# Autodesk Inventor assembly: LIA0004 XILINX SHELF ASSY
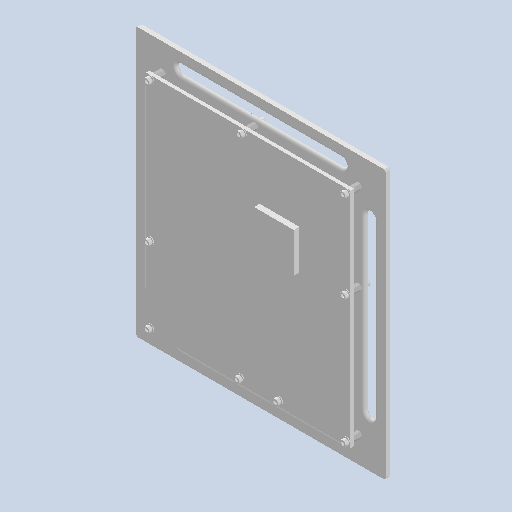
[picture p0: Inventor's stored thumbnail of the model, 512x512]
Saved by Autodesk Inventor 2023 (Build 270158000, 158)
## iProperties
Created: 2023-04-03
Part Number: LIA0004 XILINX SHELF ASSY
Document SubType Name: Assembly
Designer: Louis
Author: Louis
## Documents named in this file (7)
- D:\Louis\Documents\Inventor\Interferometry\LIA0004-XILINX SHELF ASSY.iam
- D:\Louis\Documents\Inventor\Interferometry\LI0009-XILINX SHELF.ipt
- D:\Louis\Documents\Inventor\Interferometry\XILINX BOARD FOOTPRINT.ipt
- D:\Louis\Documents\Inventor\Interferometry\ACCU HHTPS-M3-5-8-S-Z.ipt
- D:\Louis\Documents\Inventor\Interferometry\M3 WASHER.ipt
- D:\Louis\Documents\Inventor\Interferometry\M3 X 6.ipt
- D:\Louis\Documents\Inventor\Interferometry\XCZU48DR-FFVE1156 DIE.ipt
## Components (48 placed, 6 different names)
1. LI0009-XILINX SHELF:1 — Mate:1, Mate:2, Mate:3, Mate:4, Insert:1, Insert:2, Insert:3, Insert:4, Insert:5, Insert:6, Insert:7, Insert:8, Angle:1, Angle:2, Angle:3, Angle:4, Angle:5, Angle:6, Angle:7, Angle:8, Angle:9, Insert:27, Insert:28, Insert:29, Insert:30, Insert:31, Insert:32, Insert:33, Insert:34, Insert:35
2. XILINX BOARD FOOTPRINT:1 — Insert:9, Insert:10, Insert:11, Insert:12, Insert:13, Insert:14, Insert:15, Insert:16, Insert:17, Insert:18, Insert:19, Insert:20, Insert:21, Insert:22, Insert:23, Insert:24, Insert:25, Insert:26, Mate:5, Flush:1, Flush:2
3. ACCU HHTPS-M3-5-8-S-Z:1 — Mate:4, Insert:15, Angle:4
4. ACCU HHTPS-M3-5-8-S-Z:2 — Insert:1, Insert:16, Angle:3
5. ACCU HHTPS-M3-5-8-S-Z:3 — Insert:2, Insert:17, Angle:2
6. ACCU HHTPS-M3-5-8-S-Z:4 — Insert:3, Insert:9, Angle:1
7. ACCU HHTPS-M3-5-8-S-Z:6 — Insert:8, Insert:14, Angle:5
8. ACCU HHTPS-M3-5-8-S-Z:7 — Insert:7, Insert:13, Angle:6
9. ACCU HHTPS-M3-5-8-S-Z:8 — Insert:6, Insert:12, Angle:7
10. ACCU HHTPS-M3-5-8-S-Z:9 — Insert:5, Insert:11, Angle:9
11. ACCU HHTPS-M3-5-8-S-Z:10 — Insert:4, Insert:10, Angle:8
12. M3 WASHER:1 — Insert:21, Insert:41
13. M3 WASHER:2 — Insert:20, Insert:40
14. M3 WASHER:3 — Insert:23, Insert:43
15. M3 WASHER:4 — Insert:22, Insert:42
16. M3 WASHER:5 — Insert:19, Insert:39
17. M3 WASHER:6 — Insert:18, Insert:38
18. M3 WASHER:7 — Insert:25, Insert:36
19. M3 WASHER:8 — Insert:26, Insert:37
20. M3 WASHER:9 — Insert:27, Insert:45
21. M3 WASHER:10 — Insert:24, Insert:44
22. M3 WASHER:11 — Insert:35, Insert:46
23. M3 WASHER:12 — Insert:34, Insert:47
24. M3 WASHER:13 — Insert:33, Insert:48
25. M3 WASHER:14 — Insert:31, Insert:50
26. M3 WASHER:15 — Insert:32, Insert:49
27. M3 WASHER:16 — Insert:30, Insert:51
28. M3 WASHER:17 — Insert:29, Insert:52
29. M3 WASHER:18 — Insert:28, Insert:53
30. M3 X 6:1 — Insert:51
31. M3 X 6:2 — Insert:45
32. M3 X 6:3 — Insert:37
33. M3 X 6:4 — Insert:43
34. M3 X 6:5 — Insert:36
35. M3 X 6:6 — Insert:38
36. M3 X 6:7 — Insert:53
37. M3 X 6:8 — Insert:49
38. M3 X 6:9 — Insert:50
39. M3 X 6:10 — Insert:52
40. M3 X 6:11 — Insert:46
41. M3 X 6:12 — Insert:39
42. M3 X 6:13 — Insert:44
43. M3 X 6:14 — Insert:42
44. M3 X 6:15 — Insert:40
45. M3 X 6:16 — Insert:41
46. M3 X 6:17 — Insert:48
47. M3 X 6:18 — Insert:47
48. XCZU48DR-FFVE1156 DIE:1 — Mate:5, Flush:1, Flush:2
## Relationships (69: Insert 53, Angle 9, Mate 5, Flush 2)
- Mate:1: LI0009-XILINX SHELF:1
- Mate:2: LI0009-XILINX SHELF:1
- Mate:3: LI0009-XILINX SHELF:1
- Mate:4: LI0009-XILINX SHELF:1 ↔ ACCU HHTPS-M3-5-8-S-Z:1
- Insert:1: LI0009-XILINX SHELF:1 ↔ ACCU HHTPS-M3-5-8-S-Z:2
- Insert:2: LI0009-XILINX SHELF:1 ↔ ACCU HHTPS-M3-5-8-S-Z:3
- Insert:3: LI0009-XILINX SHELF:1 ↔ ACCU HHTPS-M3-5-8-S-Z:4
- Insert:4: LI0009-XILINX SHELF:1 ↔ ACCU HHTPS-M3-5-8-S-Z:10
- Insert:5: LI0009-XILINX SHELF:1 ↔ ACCU HHTPS-M3-5-8-S-Z:9
- Insert:6: LI0009-XILINX SHELF:1 ↔ ACCU HHTPS-M3-5-8-S-Z:8
- Insert:7: LI0009-XILINX SHELF:1 ↔ ACCU HHTPS-M3-5-8-S-Z:7
- Insert:8: LI0009-XILINX SHELF:1 ↔ ACCU HHTPS-M3-5-8-S-Z:6
- Insert:9: XILINX BOARD FOOTPRINT:1 ↔ ACCU HHTPS-M3-5-8-S-Z:4
- Insert:10: XILINX BOARD FOOTPRINT:1 ↔ ACCU HHTPS-M3-5-8-S-Z:10
- Insert:11: XILINX BOARD FOOTPRINT:1 ↔ ACCU HHTPS-M3-5-8-S-Z:9
- Insert:12: XILINX BOARD FOOTPRINT:1 ↔ ACCU HHTPS-M3-5-8-S-Z:8
- Insert:13: XILINX BOARD FOOTPRINT:1 ↔ ACCU HHTPS-M3-5-8-S-Z:7
- Insert:14: XILINX BOARD FOOTPRINT:1 ↔ ACCU HHTPS-M3-5-8-S-Z:6
- Insert:15: XILINX BOARD FOOTPRINT:1 ↔ ACCU HHTPS-M3-5-8-S-Z:1
- Insert:16: XILINX BOARD FOOTPRINT:1 ↔ ACCU HHTPS-M3-5-8-S-Z:2
- Insert:17: XILINX BOARD FOOTPRINT:1 ↔ ACCU HHTPS-M3-5-8-S-Z:3
- Angle:1 (0 deg): LI0009-XILINX SHELF:1 ↔ ACCU HHTPS-M3-5-8-S-Z:4
- Angle:2 (0 deg): LI0009-XILINX SHELF:1 ↔ ACCU HHTPS-M3-5-8-S-Z:3
- Angle:3 (0 deg): LI0009-XILINX SHELF:1 ↔ ACCU HHTPS-M3-5-8-S-Z:2
- Angle:4 (0 deg): LI0009-XILINX SHELF:1 ↔ ACCU HHTPS-M3-5-8-S-Z:1
- Angle:5 (0 deg): LI0009-XILINX SHELF:1 ↔ ACCU HHTPS-M3-5-8-S-Z:6
- Angle:6 (0 deg): LI0009-XILINX SHELF:1 ↔ ACCU HHTPS-M3-5-8-S-Z:7
- Angle:7 (0 deg): LI0009-XILINX SHELF:1 ↔ ACCU HHTPS-M3-5-8-S-Z:8
- Angle:8 (0 deg): LI0009-XILINX SHELF:1 ↔ ACCU HHTPS-M3-5-8-S-Z:10
- Angle:9 (0 deg): LI0009-XILINX SHELF:1 ↔ ACCU HHTPS-M3-5-8-S-Z:9
- Insert:18: XILINX BOARD FOOTPRINT:1 ↔ M3 WASHER:6
- Insert:19: XILINX BOARD FOOTPRINT:1 ↔ M3 WASHER:5
- Insert:20: XILINX BOARD FOOTPRINT:1 ↔ M3 WASHER:2
- Insert:21: XILINX BOARD FOOTPRINT:1 ↔ M3 WASHER:1
- Insert:22: XILINX BOARD FOOTPRINT:1 ↔ M3 WASHER:4
- Insert:23: XILINX BOARD FOOTPRINT:1 ↔ M3 WASHER:3
- Insert:24: XILINX BOARD FOOTPRINT:1 ↔ M3 WASHER:10
- Insert:25: XILINX BOARD FOOTPRINT:1 ↔ M3 WASHER:7
- Insert:26: XILINX BOARD FOOTPRINT:1 ↔ M3 WASHER:8
- Insert:27: LI0009-XILINX SHELF:1 ↔ M3 WASHER:9
- Insert:28: LI0009-XILINX SHELF:1 ↔ M3 WASHER:18
- Insert:29: LI0009-XILINX SHELF:1 ↔ M3 WASHER:17
- Insert:30: LI0009-XILINX SHELF:1 ↔ M3 WASHER:16
- Insert:31: LI0009-XILINX SHELF:1 ↔ M3 WASHER:14
- Insert:32: LI0009-XILINX SHELF:1 ↔ M3 WASHER:15
- Insert:33: LI0009-XILINX SHELF:1 ↔ M3 WASHER:13
- Insert:34: LI0009-XILINX SHELF:1 ↔ M3 WASHER:12
- Insert:35: LI0009-XILINX SHELF:1 ↔ M3 WASHER:11
- Insert:36: M3 WASHER:7 ↔ M3 X 6:5
- Insert:37: M3 WASHER:8 ↔ M3 X 6:3
- Insert:38: M3 WASHER:6 ↔ M3 X 6:6
- Insert:39: M3 WASHER:5 ↔ M3 X 6:12
- Insert:40: M3 WASHER:2 ↔ M3 X 6:15
- Insert:41: M3 WASHER:1 ↔ M3 X 6:16
- Insert:42: M3 WASHER:4 ↔ M3 X 6:14
- Insert:43: M3 WASHER:3 ↔ M3 X 6:4
- Insert:44: M3 WASHER:10 ↔ M3 X 6:13
- Insert:45: M3 WASHER:9 ↔ M3 X 6:2
- Insert:46: M3 WASHER:11 ↔ M3 X 6:11
- Insert:47: M3 WASHER:12 ↔ M3 X 6:18
- Insert:48: M3 WASHER:13 ↔ M3 X 6:17
- Insert:49: M3 WASHER:15 ↔ M3 X 6:8
- Insert:50: M3 WASHER:14 ↔ M3 X 6:9
- Insert:51: M3 WASHER:16 ↔ M3 X 6:1
- Insert:52: M3 WASHER:17 ↔ M3 X 6:10
- Insert:53: M3 WASHER:18 ↔ M3 X 6:7
- Mate:5: XILINX BOARD FOOTPRINT:1 ↔ XCZU48DR-FFVE1156 DIE:1
- Flush:1 (50 mm): XILINX BOARD FOOTPRINT:1 ↔ XCZU48DR-FFVE1156 DIE:1
- Flush:2 (100 mm): XILINX BOARD FOOTPRINT:1 ↔ XCZU48DR-FFVE1156 DIE:1
